# Autodesk Inventor assembly: Male_Tail_Female_Connector(final)
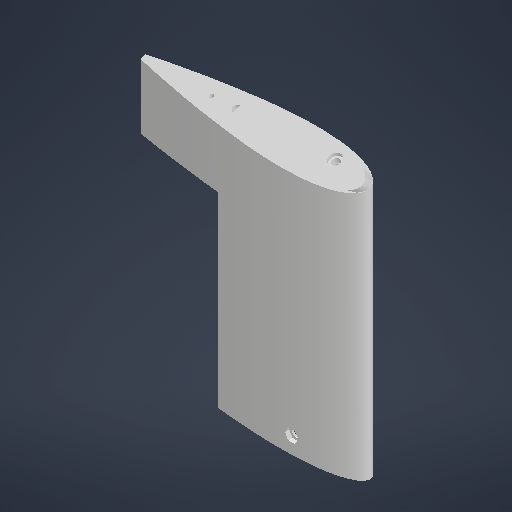
[picture p0: Inventor's stored thumbnail of the model, 512x512]
Saved by Autodesk Inventor 2026 (Build 300175050, 175E)
## iProperties
Created: 2026-07-13
Part Number: Male_Tail_Female_Connector(final)
Document SubType Name: Assembly
Designer: Delbe
Author: Delbe
## Documents named in this file (3)
- C:\GitHub\SWIFT-UAV\System_development\Pelican\structural_model\v0.3.0\Parts\Delb_Parts\Male_Tail_Female_Connector(final).iam
- C:\GitHub\SWIFT-UAV\System_development\Pelican\structural_model\v0.3.0\Parts\Delb_Parts\Male_Tail_Female_Connector.ipt
- C:\GitHub\SWIFT-UAV\System_development\Pelican\structural_model\v0.3.0\Parts\Delb_Parts\connector.ipt
## Components (2 placed, 2 different names)
1. Male_Tail_Female_Connector:1 — Rigid:1
2. connector:1 — Rigid:1
## Relationships (1: WeldJoint 1)
- Rigid:1 [WeldJoint]: Male_Tail_Female_Connector:1 ↔ connector:1
